# Autodesk Inventor assembly: World
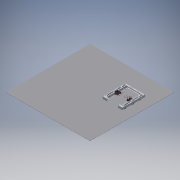
[picture p0: Inventor's stored thumbnail of the model, 180x180]
Saved by Autodesk Inventor 2019 (Build 230136000, 136)
## iProperties
Created: 2020-01-13
Part Number: World
Document SubType Name: Assembly
Designer: james
Author: james
## Documents named in this file (3)
- F:\JimsRobot\FIRSTRobots\Design\JimsCHS2020FRC\World.iam
- F:\JimsRobot\FIRSTRobots\Design\JimsCHS2020FRC\DriveBase.iam
- F:\JimsRobot\FIRSTRobots\Design\Library\Jims\Carpet.ipt
## Components (2 placed, 2 different names)
1. DriveBase:1 [sub-assembly] — Mate:1
2. Carpet:1 — Mate:1
## Relationships (1: Mate 1)
- Mate:1 (48.26 mm): DriveBase:1 ↔ Carpet:1
